# Autodesk Inventor assembly: NP18-12
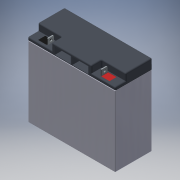
[picture p0: Inventor's stored thumbnail of the model, 180x180]
Saved by Autodesk Inventor 2017.1 (Build 211199000, 199)
## iProperties
Company: Autodesk Inc.
Created: 2016-12-23
Part Number: NP18-12
Document SubType Name: Assembly
Designer: Autodesk
Description: Battery, ,12 volt, 18 AH, Non-spillable
Catalog Web Link: http://www.enersys.com/default.aspx?langType=1033
Vendor: EnerSys
Author: Autodesk Inc.
Keywords: Separate Items
## Documents named in this file (3)
- D:\FIRST\FIRST KOP 2017\FIRST 2017 Separate Items\NP18-12.iam
- D:\FIRST\FIRST KOP 2017\FIRST 2017 Separate Items\Parts\Electrical_Yuasa_NP18-12_Top.ipt
- D:\FIRST\FIRST KOP 2017\FIRST 2017 Separate Items\Parts\Electrical_Yuasa_Np18-12_Middle.ipt
## Components (2 placed, 2 different names)
1. Electrical_Yuasa_NP18-12_Top:1 — Flush:1
2. Electrical_Yuasa_Np18-12_Middle:1 — Flush:1
## Relationships (1: Flush 1)
- Flush:1: Electrical_Yuasa_NP18-12_Top:1 ↔ Electrical_Yuasa_Np18-12_Middle:1
